# Autodesk Inventor assembly: гроб для задницы цел нормис_MIR
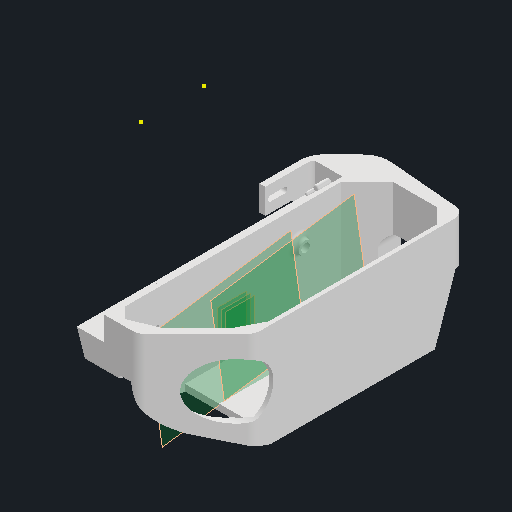
[picture p0: Inventor's stored thumbnail of the model, 512x512]
Saved by Autodesk Inventor 2025 (Build 290162000, 162)
## iProperties
Created: 2024-09-20
Part Number: гроб для задницы цел нормис_MIR
Document SubType Name: Assembly
Designer: GameHD
Author: GameHD
## Documents named in this file (3)
- C:\Users\GameHD\Desktop\что-то нужное\Phantom16950\гроб для задницы цел нормис_MIR.iam
- C:\Users\GameHD\Desktop\что-то нужное\Phantom16950\гроб для задницы нормис 2Ч_MIR.ipt
- C:\Users\GameHD\Desktop\что-то нужное\Phantom16950\гроб для задницы нормис_MIR.ipt
## Components (2 placed, 2 different names)
1. гроб для задницы нормис 2Ч_MIR:1 — Заподлицо:2, Заподлицо:1, Совмещение:1
2. гроб для задницы нормис_MIR:1 — Заподлицо:2, Заподлицо:1, Совмещение:1
## Relationships (3: Flush 2, Mate 1)
- Заподлицо:2 [Flush]: гроб для задницы нормис 2Ч_MIR:1 ↔ гроб для задницы нормис_MIR:1
- Заподлицо:1 [Flush]: гроб для задницы нормис 2Ч_MIR:1 ↔ гроб для задницы нормис_MIR:1
- Совмещение:1 [Mate]: гроб для задницы нормис 2Ч_MIR:1 ↔ гроб для задницы нормис_MIR:1
